# Autodesk Inventor assembly: MCU_PCB
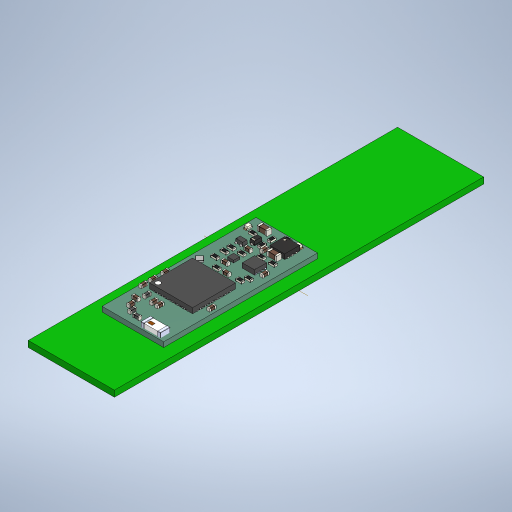
[picture p0: Inventor's stored thumbnail of the model, 512x512]
Saved by Autodesk Inventor 2024 (Build 280153000, 153)
## iProperties
Created: 2025-02-15
Part Number: MCU_PCB
Document SubType Name: Assembly
Designer: XxPan
Author: XxPan
## Documents named in this file (3)
- C:\Users\XxPan\OneDrive - McMaster University\4OI6\InkSync\case\MCU_PCB.iam
- C:\Users\XxPan\OneDrive - McMaster University\4OI6\InkSync\case\MCU_PCB.ipt
- C:\Users\XxPan\OneDrive - McMaster University\4OI6\InkSync\case\OMGS3\OMGS3.iam
## Components (2 placed, 2 different names)
1. MCU_PCB:1 — Mate:1, Angle:1, Flush:1, Flush:2
2. OMGS3:1 [sub-assembly] — Mate:1, Angle:1, Flush:1, Flush:2
## Relationships (4: Flush 2, Mate 1, Angle 1)
- Mate:1: MCU_PCB:1 ↔ OMGS3:1
- Angle:1 (0 deg): MCU_PCB:1 ↔ OMGS3:1
- Flush:1 (2 mm): MCU_PCB:1 ↔ OMGS3:1
- Flush:2 (10 mm): MCU_PCB:1 ↔ OMGS3:1
